# Autodesk Inventor assembly: holding the motor
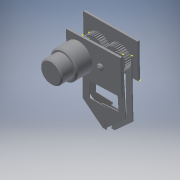
[picture p0: Inventor's stored thumbnail of the model, 180x180]
Saved by Autodesk Inventor 2019 (Build 230136000, 136)
## iProperties
Created: 2020-03-03
Part Number: holding the motor
Document SubType Name: Assembly
Designer: VIGNESH
Author: VIGNESH
## Documents named in this file (8)
- C:\Users\VIGNESH\Documents\holding the motor.iam
- C:\Users\VIGNESH\Documents\motor 2.ipt
- C:\Users\VIGNESH\Documents\motor bolt.ipt
- C:\Users\VIGNESH\Documents\robotic arm fixer.ipt
- C:\Users\VIGNESH\Documents\now1.iam
- C:\Users\VIGNESH\Documents\5mm bolt 40 mm height.ipt
- C:\Users\VIGNESH\Documents\5mm fixer.ipt
- C:\Users\VIGNESH\Documents\gripper holder.ipt
## Components (10 placed, 7 different names)
1. motor 2:1 — Rotational:1, Rotational:2, Rotational:3
2. motor bolt:1 — Rotational:2
3. robotic arm fixer:1 — Rotational:1, Mate:1
4. now1:1 [sub-assembly] — Rotational:3, Mate:1, Rotational:4, Mate:2, Mate:3
5. 5mm bolt 40 mm height:1 — Rotational:4, Rotational:5
6. 5mm fixer:1 — Rotational:5
7. gripper holder:1
8. gripper holder:2
9. gripper holder:3 — Mate:2
10. gripper holder:4 — Mate:3
## Relationships (8: RevoluteJoint 5, Mate 3)
- Rotational:1 [RevoluteJoint] (-5 mm): motor 2:1 ↔ robotic arm fixer:1
- Rotational:2 [RevoluteJoint] (-1 mm): motor 2:1 ↔ motor bolt:1
- Rotational:3 [RevoluteJoint] (20 mm): motor 2:1 ↔ now1:1
- Mate:1: robotic arm fixer:1 ↔ now1:1
- Rotational:4 [RevoluteJoint] (40 mm): now1:1 ↔ 5mm bolt 40 mm height:1
- Rotational:5 [RevoluteJoint]: 5mm bolt 40 mm height:1 ↔ 5mm fixer:1
- Mate:2: now1:1 ↔ gripper holder:3
- Mate:3: now1:1 ↔ gripper holder:4
